# Autodesk Inventor assembly: Tensionador-3-Cabos_Modelo2
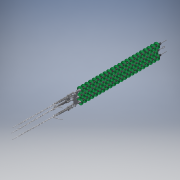
[picture p0: Inventor's stored thumbnail of the model, 180x180]
Saved by Autodesk Inventor 2018 (Build 220112000, 112)
## iProperties
Created: 2021-08-02
Part Number: Tensionador-3-Cabos_Modelo2
Document SubType Name: Assembly
Designer: L08619
Author: L08619
## Documents named in this file (6)
- F:\Projetos\TAESA\Modelo 3D - Tensionadores e Suspensão\Tensionador\Tensionador-3-Cabos_Modelo2.iam
- F:\Projetos\TAESA\Modelo 3D - Tensionadores e Suspensão\Tensionador\Balancim_3-Cabos_Modelo2.ipt
- F:\Projetos\TAESA\Modelo 3D - Tensionadores e Suspensão\Tensionador\Clevis-Socket.iam
- F:\Projetos\TAESA\Modelo 3D - Tensionadores e Suspensão\Tensionador\gpghmb32.iam
- F:\Projetos\TAESA\Modelo 3D - Tensionadores e Suspensão\Tensionador\OPGW Tension set.iam
- F:\Projetos\TAESA\Modelo 3D - Tensionadores e Suspensão\Suporte de Suspenção\Suspensao.ipt
## Components (16 placed, 5 different names)
1. Balancim_3-Cabos_Modelo2:1 — Mate:1, Mate:2, Cylindrical:2, Cylindrical:4, Cylindrical:5, Cylindrical:6, Mate:4, Mate:6, Mate:7, Mate:8, Mate:9, Cylindrical:7, Cylindrical:8, Mate:10
2. Clevis-Socket:1 [sub-assembly] — Mate:9, Cylindrical:7, Rigid:3
3. Clevis-Socket:2 [sub-assembly] — Cylindrical:2, Mate:4, Rigid:2
4. Clevis-Socket:3 [sub-assembly] — Cylindrical:8, Mate:10, Rigid:1
5. gpghmb32:1 [sub-assembly] — Cylindrical:5, Mate:8
6. gpghmb32:3 [sub-assembly] — Cylindrical:6, Mate:7
7. gpghmb32:4 [sub-assembly] — Cylindrical:4, Mate:6
8. gpghmb32:5 [sub-assembly] — Mate:11, Rotational:1, Angle:2
9. gpghmb32:6 [sub-assembly] — Mate:12, Rotational:3, Angle:3
10. gpghmb32:7 [sub-assembly] — Rotational:2
11. OPGW Tension set:2 [sub-assembly] — Rotational:1
12. OPGW Tension set:3 [sub-assembly] — Rotational:2, Angle:1
13. OPGW Tension set:4 [sub-assembly] — Rotational:3
14. Suspensao:1 — Rigid:2
15. Suspensao:2 — Rigid:1
16. Suspensao:3 — Rigid:3
## Relationships (25: Mate 10, CylindricalJoint 6, RevoluteJoint 3, Angle 3, WeldJoint 3)
- Mate:1: Balancim_3-Cabos_Modelo2:1
- Mate:2: Balancim_3-Cabos_Modelo2:1
- Cylindrical:2: Balancim_3-Cabos_Modelo2:1 ↔ Clevis-Socket:2
- Cylindrical:4: Balancim_3-Cabos_Modelo2:1 ↔ gpghmb32:4
- Cylindrical:5: Balancim_3-Cabos_Modelo2:1 ↔ gpghmb32:1
- Cylindrical:6: Balancim_3-Cabos_Modelo2:1 ↔ gpghmb32:3
- Mate:4 (2 mm): Balancim_3-Cabos_Modelo2:1 ↔ Clevis-Socket:2
- Mate:6 (10 mm): Balancim_3-Cabos_Modelo2:1 ↔ gpghmb32:4
- Mate:7 (10 mm): Balancim_3-Cabos_Modelo2:1 ↔ gpghmb32:3
- Mate:8 (10 mm): Balancim_3-Cabos_Modelo2:1 ↔ gpghmb32:1
- Mate:9 (2 mm): Balancim_3-Cabos_Modelo2:1 ↔ Clevis-Socket:1
- Cylindrical:7: Balancim_3-Cabos_Modelo2:1 ↔ Clevis-Socket:1
- Cylindrical:8: Balancim_3-Cabos_Modelo2:1 ↔ Clevis-Socket:3
- Mate:10 (2 mm): Balancim_3-Cabos_Modelo2:1 ↔ Clevis-Socket:3
- Mate:11: gpghmb32:5
- Mate:12: gpghmb32:6
- Rotational:1 [RevoluteJoint]: gpghmb32:5 ↔ OPGW Tension set:2
- Rotational:2 [RevoluteJoint]: gpghmb32:7 ↔ OPGW Tension set:3
- Rotational:3 [RevoluteJoint]: gpghmb32:6 ↔ OPGW Tension set:4
- Angle:1 (270 deg): OPGW Tension set:3
- Angle:2 (0 deg): gpghmb32:5
- Angle:3 (0 deg): gpghmb32:6
- Rigid:1 [WeldJoint]: Clevis-Socket:3 ↔ Suspensao:2
- Rigid:2 [WeldJoint]: Clevis-Socket:2 ↔ Suspensao:1
- Rigid:3 [WeldJoint]: Clevis-Socket:1 ↔ Suspensao:3
